# Autodesk Inventor assembly: Retro PC
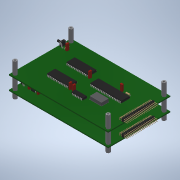
[picture p0: Inventor's stored thumbnail of the model, 180x180]
Saved by Autodesk Inventor 2020.2 (Build 242310000, 310)
## iProperties
Created: 2019-12-02
Part Number: Retro PC
Material: Generisch
Document SubType Name: Assembly
Designer: Daniel
Author: Daniel
## Documents named in this file (5)
- C:\Users\Daniel.Kampert\Desktop\Git\Retro PC\drawing\Retro PC.iam
- C:\Users\Daniel.Kampert\Desktop\Git\Retro PC\export\PowerSupply.ipt
- C:\Users\Daniel.Kampert\Desktop\Git\Retro PC\export\ProcessorBoardProcessorBoard.ipt
- C:\Users\Daniel.Kampert\Desktop\Git\Retro PC\export\WUERTH 449843 20 spacer stud BLZ-ABSTAND-ST-I_A-SW5,5-A2K-M3X20-7-6.ipt
- C:\Users\Daniel.Kampert\Desktop\Git\Retro PC\export\WUERTH 449863 10 spacer stud BLZ-ABSTAND-ST-I_I-SW5,5-A2K-M3X10-10.ipt
## Components (14 placed, 4 different names)
1. PowerSupply:1 — Passend:20, Passend:21, Passend:22, Passend:27, Passend:28, Passend:29, Passend:30, Passend:31, Passend:32, Passend:33, Passend:34, Passend:35
2. ProcessorBoardProcessorBoard:1 — Passend:6, Passend:7, Passend:8, Passend:9, Passend:10, Passend:11, Passend:12, Passend:14, Passend:15, Passend:23, Passend:24, Passend:25, Passend:26
3. WUERTH 449843 20 spacer stud BLZ-ABSTAND-ST-I_A-SW5,5-A2K-M3X20-7-6:1 — Passend:25, Passend:26
4. WUERTH 449863 10 spacer stud BLZ-ABSTAND-ST-I_I-SW5,5-A2K-M3X10-10:1 — Passend:32, Passend:36
5. WUERTH 449863 10 spacer stud BLZ-ABSTAND-ST-I_I-SW5,5-A2K-M3X10-10:2 — Passend:33, Passend:37
6. WUERTH 449863 10 spacer stud BLZ-ABSTAND-ST-I_I-SW5,5-A2K-M3X10-10:3 — Passend:34, Passend:39
7. WUERTH 449863 10 spacer stud BLZ-ABSTAND-ST-I_I-SW5,5-A2K-M3X10-10:4 — Passend:35, Passend:38
8. WUERTH 449843 20 spacer stud BLZ-ABSTAND-ST-I_A-SW5,5-A2K-M3X20-7-6:2 — Passend:6, Passend:10, Passend:13
9. WUERTH 449843 20 spacer stud BLZ-ABSTAND-ST-I_A-SW5,5-A2K-M3X20-7-6:3 — Passend:7, Passend:11, Passend:18
10. WUERTH 449843 20 spacer stud BLZ-ABSTAND-ST-I_A-SW5,5-A2K-M3X20-7-6:4 — Passend:8, Passend:9, Passend:19
11. WUERTH 449843 20 spacer stud BLZ-ABSTAND-ST-I_A-SW5,5-A2K-M3X20-7-6:5 — Passend:12, Passend:13, Passend:22, Passend:31, Passend:36
12. WUERTH 449843 20 spacer stud BLZ-ABSTAND-ST-I_A-SW5,5-A2K-M3X20-7-6:6 — Passend:14, Passend:19, Passend:20, Passend:29, Passend:39
13. WUERTH 449843 20 spacer stud BLZ-ABSTAND-ST-I_A-SW5,5-A2K-M3X20-7-6:7 — Passend:23, Passend:24, Passend:27, Passend:28, Passend:37
14. WUERTH 449843 20 spacer stud BLZ-ABSTAND-ST-I_A-SW5,5-A2K-M3X20-7-6:8 — Passend:15, Passend:18, Passend:21, Passend:30, Passend:38
## Relationships (32: Mate 32)
- Passend:6 [Mate]: ProcessorBoardProcessorBoard:1 ↔ WUERTH 449843 20 spacer stud BLZ-ABSTAND-ST-I_A-SW5,5-A2K-M3X20-7-6:2
- Passend:7 [Mate]: ProcessorBoardProcessorBoard:1 ↔ WUERTH 449843 20 spacer stud BLZ-ABSTAND-ST-I_A-SW5,5-A2K-M3X20-7-6:3
- Passend:8 [Mate]: ProcessorBoardProcessorBoard:1 ↔ WUERTH 449843 20 spacer stud BLZ-ABSTAND-ST-I_A-SW5,5-A2K-M3X20-7-6:4
- Passend:9 [Mate]: ProcessorBoardProcessorBoard:1 ↔ WUERTH 449843 20 spacer stud BLZ-ABSTAND-ST-I_A-SW5,5-A2K-M3X20-7-6:4
- Passend:10 [Mate]: ProcessorBoardProcessorBoard:1 ↔ WUERTH 449843 20 spacer stud BLZ-ABSTAND-ST-I_A-SW5,5-A2K-M3X20-7-6:2
- Passend:11 [Mate]: ProcessorBoardProcessorBoard:1 ↔ WUERTH 449843 20 spacer stud BLZ-ABSTAND-ST-I_A-SW5,5-A2K-M3X20-7-6:3
- Passend:12 [Mate]: ProcessorBoardProcessorBoard:1 ↔ WUERTH 449843 20 spacer stud BLZ-ABSTAND-ST-I_A-SW5,5-A2K-M3X20-7-6:5
- Passend:13 [Mate]: WUERTH 449843 20 spacer stud BLZ-ABSTAND-ST-I_A-SW5,5-A2K-M3X20-7-6:2 ↔ WUERTH 449843 20 spacer stud BLZ-ABSTAND-ST-I_A-SW5,5-A2K-M3X20-7-6:5
- Passend:14 [Mate]: ProcessorBoardProcessorBoard:1 ↔ WUERTH 449843 20 spacer stud BLZ-ABSTAND-ST-I_A-SW5,5-A2K-M3X20-7-6:6
- Passend:15 [Mate]: ProcessorBoardProcessorBoard:1 ↔ WUERTH 449843 20 spacer stud BLZ-ABSTAND-ST-I_A-SW5,5-A2K-M3X20-7-6:8
- Passend:18 [Mate]: WUERTH 449843 20 spacer stud BLZ-ABSTAND-ST-I_A-SW5,5-A2K-M3X20-7-6:3 ↔ WUERTH 449843 20 spacer stud BLZ-ABSTAND-ST-I_A-SW5,5-A2K-M3X20-7-6:8
- Passend:19 [Mate]: WUERTH 449843 20 spacer stud BLZ-ABSTAND-ST-I_A-SW5,5-A2K-M3X20-7-6:4 ↔ WUERTH 449843 20 spacer stud BLZ-ABSTAND-ST-I_A-SW5,5-A2K-M3X20-7-6:6
- Passend:20 [Mate]: PowerSupply:1 ↔ WUERTH 449843 20 spacer stud BLZ-ABSTAND-ST-I_A-SW5,5-A2K-M3X20-7-6:6
- Passend:21 [Mate]: PowerSupply:1 ↔ WUERTH 449843 20 spacer stud BLZ-ABSTAND-ST-I_A-SW5,5-A2K-M3X20-7-6:8
- Passend:22 [Mate]: PowerSupply:1 ↔ WUERTH 449843 20 spacer stud BLZ-ABSTAND-ST-I_A-SW5,5-A2K-M3X20-7-6:5
- Passend:23 [Mate]: ProcessorBoardProcessorBoard:1 ↔ WUERTH 449843 20 spacer stud BLZ-ABSTAND-ST-I_A-SW5,5-A2K-M3X20-7-6:7
- Passend:24 [Mate]: ProcessorBoardProcessorBoard:1 ↔ WUERTH 449843 20 spacer stud BLZ-ABSTAND-ST-I_A-SW5,5-A2K-M3X20-7-6:7
- Passend:25 [Mate]: ProcessorBoardProcessorBoard:1 ↔ WUERTH 449843 20 spacer stud BLZ-ABSTAND-ST-I_A-SW5,5-A2K-M3X20-7-6:1
- Passend:26 [Mate]: ProcessorBoardProcessorBoard:1 ↔ WUERTH 449843 20 spacer stud BLZ-ABSTAND-ST-I_A-SW5,5-A2K-M3X20-7-6:1
- Passend:27 [Mate]: PowerSupply:1 ↔ WUERTH 449843 20 spacer stud BLZ-ABSTAND-ST-I_A-SW5,5-A2K-M3X20-7-6:7
- Passend:28 [Mate]: PowerSupply:1 ↔ WUERTH 449843 20 spacer stud BLZ-ABSTAND-ST-I_A-SW5,5-A2K-M3X20-7-6:7
- Passend:29 [Mate]: PowerSupply:1 ↔ WUERTH 449843 20 spacer stud BLZ-ABSTAND-ST-I_A-SW5,5-A2K-M3X20-7-6:6
- Passend:30 [Mate]: PowerSupply:1 ↔ WUERTH 449843 20 spacer stud BLZ-ABSTAND-ST-I_A-SW5,5-A2K-M3X20-7-6:8
- Passend:31 [Mate]: PowerSupply:1 ↔ WUERTH 449843 20 spacer stud BLZ-ABSTAND-ST-I_A-SW5,5-A2K-M3X20-7-6:5
- Passend:32 [Mate]: PowerSupply:1 ↔ WUERTH 449863 10 spacer stud BLZ-ABSTAND-ST-I_I-SW5,5-A2K-M3X10-10:1
- Passend:33 [Mate]: PowerSupply:1 ↔ WUERTH 449863 10 spacer stud BLZ-ABSTAND-ST-I_I-SW5,5-A2K-M3X10-10:2
- Passend:34 [Mate]: PowerSupply:1 ↔ WUERTH 449863 10 spacer stud BLZ-ABSTAND-ST-I_I-SW5,5-A2K-M3X10-10:3
- Passend:35 [Mate]: PowerSupply:1 ↔ WUERTH 449863 10 spacer stud BLZ-ABSTAND-ST-I_I-SW5,5-A2K-M3X10-10:4
- Passend:36 [Mate]: WUERTH 449863 10 spacer stud BLZ-ABSTAND-ST-I_I-SW5,5-A2K-M3X10-10:1 ↔ WUERTH 449843 20 spacer stud BLZ-ABSTAND-ST-I_A-SW5,5-A2K-M3X20-7-6:5
- Passend:37 [Mate]: WUERTH 449863 10 spacer stud BLZ-ABSTAND-ST-I_I-SW5,5-A2K-M3X10-10:2 ↔ WUERTH 449843 20 spacer stud BLZ-ABSTAND-ST-I_A-SW5,5-A2K-M3X20-7-6:7
- Passend:38 [Mate]: WUERTH 449863 10 spacer stud BLZ-ABSTAND-ST-I_I-SW5,5-A2K-M3X10-10:4 ↔ WUERTH 449843 20 spacer stud BLZ-ABSTAND-ST-I_A-SW5,5-A2K-M3X20-7-6:8
- Passend:39 [Mate]: WUERTH 449863 10 spacer stud BLZ-ABSTAND-ST-I_I-SW5,5-A2K-M3X10-10:3 ↔ WUERTH 449843 20 spacer stud BLZ-ABSTAND-ST-I_A-SW5,5-A2K-M3X20-7-6:6
